# Autodesk Inventor assembly: GFRP_T2_01
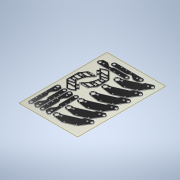
[picture p0: Inventor's stored thumbnail of the model, 180x180]
Saved by Autodesk Inventor 2022 (Build 260153000, 153)
## iProperties
Created: 2022-09-28
Part Number: GFRP_T2_01
Document SubType Name: Assembly
Designer: Masato
Author: Masato
## Documents named in this file (5)
- C:\Users\MasatoKubotera\Documents\Inventor\SUSTAINA-OP - CAM\Cam\GFRP_T2\OriginalMind_RD400\GFRP_T2_01.iam
- C:\Users\MasatoKubotera\Documents\Inventor\SUSTAINA-OP - CAM\Cam\DisposableBoard.ipt
- C:\Users\MasatoKubotera\Documents\Inventor\SUSTAINA-OP - CAM\UpperBody\Head\Head_neck_side_frame.ipt
- C:\Users\MasatoKubotera\Documents\Inventor\SUSTAINA-OP - CAM\LowerBody\Link\BackLink_frame.ipt
- C:\Users\MasatoKubotera\Documents\Inventor\SUSTAINA-OP - CAM\LowerBody\Link\FrontLink_frame.ipt
## Components (15 placed, 4 different names)
1. DisposableBoard:1 — フラッシュ:1, フラッシュ:2, フラッシュ:3, フラッシュ:4, フラッシュ:6, 正接:1, 正接:2, 正接:4, 正接:5, フラッシュ:9, 角度:2, 正接:9
2. Head_neck_side_frame:2 — メイト:14, 角度:1, 正接:7, メイト:15, 正接:8
3. Head_neck_side_frame:7 — 正接:6, メイト:13, フラッシュ:9, 角度:1, メイト:15
4. BackLink_frame:16 — メイト:10, メイト:12, 角度:2, 正接:10
5. BackLink_frame:17 — メイト:11, メイト:12, 正接:8, 正接:9
6. BackLink_frame:4 — フラッシュ:6, メイト:5, 正接:1, メイト:8
7. BackLink_frame:7 — メイト:6, 正接:2, メイト:8, 正接:6
8. BackLink_frame:14
9. BackLink_frame:15
10. FrontLink_frame:3 — メイト:9, 正接:4, 正接:5
11. FrontLink_frame:12
12. FrontLink_frame:13
13. FrontLink_frame:14
14. FrontLink_frame:15 — 正接:7
15. FrontLink_frame:16 — 正接:10
## Component patterns: (2 elements, first: BackLink_frame:4 + BackLink_frame:7), (6 elements, first: FrontLink_frame:3)
## Relationships (27: Mate 10, Tangent 9, Flush 6, Angle 2)
- フラッシュ:1 [Flush]: DisposableBoard:1
- フラッシュ:2 [Flush]: DisposableBoard:1
- フラッシュ:3 [Flush]: DisposableBoard:1
- フラッシュ:4 [Flush]: DisposableBoard:1
- フラッシュ:6 [Flush] (2 mm): DisposableBoard:1 ↔ BackLink_frame:4
- メイト:5 [Mate]: BackLink_frame:4
- メイト:6 [Mate]: BackLink_frame:7
- 正接:1 [Tangent] (2 mm): DisposableBoard:1 ↔ BackLink_frame:4
- 正接:2 [Tangent] (2 mm): DisposableBoard:1 ↔ BackLink_frame:7
- メイト:8 [Mate] (2.1 mm): BackLink_frame:4 ↔ BackLink_frame:7
- メイト:9 [Mate]: FrontLink_frame:3
- 正接:4 [Tangent] (2 mm): DisposableBoard:1 ↔ FrontLink_frame:3
- 正接:5 [Tangent] (2 mm): DisposableBoard:1 ↔ FrontLink_frame:3
- メイト:10 [Mate]: BackLink_frame:16
- メイト:11 [Mate]: BackLink_frame:17
- メイト:12 [Mate] (2.1 mm): BackLink_frame:16 ↔ BackLink_frame:17
- 正接:6 [Tangent] (2.1 mm): Head_neck_side_frame:7 ↔ BackLink_frame:7
- メイト:13 [Mate]: Head_neck_side_frame:7
- メイト:14 [Mate]: Head_neck_side_frame:2
- フラッシュ:9 [Flush] (-2 mm): DisposableBoard:1 ↔ Head_neck_side_frame:7
- 角度:1 [Angle] (180 deg): Head_neck_side_frame:2 ↔ Head_neck_side_frame:7
- 正接:7 [Tangent] (2.1 mm): Head_neck_side_frame:2 ↔ FrontLink_frame:15
- メイト:15 [Mate] (2.1 mm): Head_neck_side_frame:2 ↔ Head_neck_side_frame:7
- 正接:8 [Tangent] (2.1 mm): Head_neck_side_frame:2 ↔ BackLink_frame:17
- 角度:2 [Angle] (0 deg): DisposableBoard:1 ↔ BackLink_frame:16
- 正接:9 [Tangent] (2.1 mm): DisposableBoard:1 ↔ BackLink_frame:17
- 正接:10 [Tangent] (2.1 mm): BackLink_frame:16 ↔ FrontLink_frame:16
